# Autodesk Inventor assembly: 8WDSingleSprocket
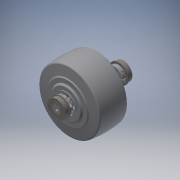
[picture p0: Inventor's stored thumbnail of the model, 180x180]
Saved by Autodesk Inventor 2016 (Build 200138000, 138)
## iProperties
Created: 2017-01-10
Part Number: 8WDSingleSprocket
Document SubType Name: Assembly
Designer: Kyle
Author: Kyle
## Documents named in this file (7)
- F:\FRC\2017\CAD Assemblies\8WDSingleSprocket.iam
- F:\FRC\2017\CAD Assemblies\.5HexShaft4.25in.ipt
- F:\FRC\2017\CAD Assemblies\.5HexBearing.ipt
- F:\FRC\2017\CAD Assemblies\.5ShaftCollar.ipt
- F:\FRC\2017\CAD Assemblies\4x2Colson.ipt
- F:\FRC\2017\CAD Assemblies\16t25Sprocket.ipt
- F:\FRC\2017\CAD Assemblies\.506Spacer.ipt
## Components (8 placed, 6 different names)
1. .5HexShaft4.25in:1 — Mate:1, Flush:1, Mate:2, Flush:2, Mate:3, Mate:5, Mate:7, Mate:9, Mate:11
2. .5HexBearing:1 — Mate:2, Flush:2, Mate:6
3. .5HexBearing:2 — Mate:1, Flush:1, Mate:4
4. .5ShaftCollar:1 — Mate:3, Mate:4, Mate:8
5. .5ShaftCollar:2 — Mate:5, Mate:6, Mate:12
6. 4x2Colson:1 — Mate:7, Mate:8, Mate:10
7. 16t25Sprocket:1 — Mate:9, Mate:10
8. .506Spacer:1 — Mate:11, Mate:12
## Relationships (14: Mate 12, Flush 2)
- Mate:1: .5HexShaft4.25in:1 ↔ .5HexBearing:2
- Flush:1: .5HexShaft4.25in:1 ↔ .5HexBearing:2
- Mate:2: .5HexShaft4.25in:1 ↔ .5HexBearing:1
- Flush:2: .5HexShaft4.25in:1 ↔ .5HexBearing:1
- Mate:3: .5HexShaft4.25in:1 ↔ .5ShaftCollar:1
- Mate:4: .5HexBearing:2 ↔ .5ShaftCollar:1
- Mate:5: .5HexShaft4.25in:1 ↔ .5ShaftCollar:2
- Mate:6: .5HexBearing:1 ↔ .5ShaftCollar:2
- Mate:7: .5HexShaft4.25in:1 ↔ 4x2Colson:1
- Mate:8: .5ShaftCollar:1 ↔ 4x2Colson:1
- Mate:9: .5HexShaft4.25in:1 ↔ 16t25Sprocket:1
- Mate:10: 4x2Colson:1 ↔ 16t25Sprocket:1
- Mate:11: .5HexShaft4.25in:1 ↔ .506Spacer:1
- Mate:12: .5ShaftCollar:2 ↔ .506Spacer:1
